# Autodesk Inventor assembly: M5 Screw with Tee Nut
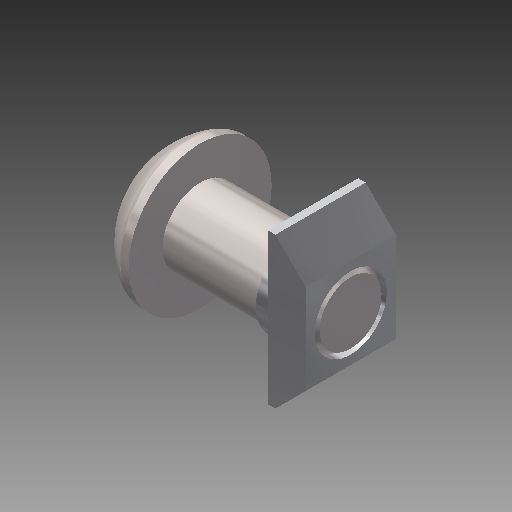
[picture p0: Inventor's stored thumbnail of the model, 512x512]
Saved by Autodesk Inventor 2017 (Build 210142000, 142)
## iProperties
Created: 2014-02-18
Part Number: M5 Screw with Tee Nut
Document SubType Name: Assembly
Designer: umr
Mass: 2.70106 g
Surface Area: 5.57941 cm^2
Volume: 0.422368 cm^3
Density: 6.39505 g/cm^3
Sending System: SolidWorks 2014
Last Author: Rory
Last Saved: 2016-05-20
Author: umr
## Documents named in this file (3)
- D:\SeniorProject\Models2\Head\M5 Screw with Tee Nut.iam
- D:\SeniorProject\Models2\Head\Tee Nut.ipt
- D:\SeniorProject\Models2\Head\M5 Screw.ipt
## Components (2 placed, 2 different names)
1. Tee Nut:1 — Mate:2, Flush:1
2. M5 Screw:1 — Mate:2, Flush:1
## Relationships (2: Mate 1, Flush 1)
- Mate:2: Tee Nut:1 ↔ M5 Screw:1
- Flush:1: Tee Nut:1 ↔ M5 Screw:1
